# Autodesk Inventor assembly: Bikair
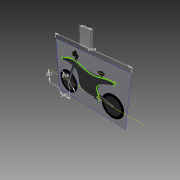
[picture p0: Inventor's stored thumbnail of the model, 180x180]
Saved by Autodesk Inventor 2014 (Build 180170000, 170)
## iProperties
Created: 2015-03-25
Part Number: Bikair
Document SubType Name: Assembly
Designer: Yann
Author: Yann
## Documents named in this file (3)
- C:\Users\Yann\Documents\GitHub\BIKAIR_CAD\Source\Bikair.iam
- C:\Users\Yann\Documents\GitHub\BIKAIR_CAD\Source\Frame\Frame.iam
- C:\Users\Yann\Documents\GitHub\BIKAIR_CAD\Source\Energy_Pack\Energy_Pack.iam
## Components (2 placed, 2 different names)
1. Frame:1 [sub-assembly] — Affleurement:1, Placage:1, Placage:2
2. Energy_Pack:1 [sub-assembly] — Affleurement:2
## Relationships (4: Flush 2, Mate 2)
- Affleurement:1 [Flush]: Frame:1
- Placage:1 [Mate]: Frame:1
- Placage:2 [Mate]: Frame:1
- Affleurement:2 [Flush]: Energy_Pack:1
